# Autodesk Inventor assembly: Assembly_4_turnsignal_MIR
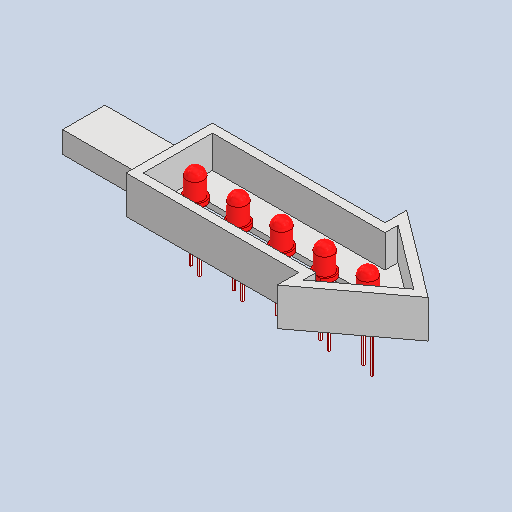
[picture p0: Inventor's stored thumbnail of the model, 512x512]
Saved by Autodesk Inventor 2023 (Build 270158000, 158)
## iProperties
Created: 2023-10-01
Part Number: Assembly_4_turnsignal_MIR
Document SubType Name: Assembly
Designer: zskus
Author: zskus
## Documents named in this file (3)
- C:\Users\zskus\Desktop\Folders\Personal Projects\Inventor\Project_1_Scooter\Assembly\Assembly_4_turnsignal_MIR.iam
- C:\Users\zskus\Desktop\Folders\Personal Projects\Inventor\Project_1_Scooter\Parts\Part_5_ledholder_MIR.ipt
- C:\Users\zskus\Desktop\Folders\Personal Projects\Inventor\Project_1_Scooter\Parts\red-led-5mm_MIR.ipt
## Components (6 placed, 2 different names)
1. Part_5_ledholder_MIR:1 — Mate:3, Mate:2, Mate:1
2. red-led-5mm_MIR:1 — Mate:3, Mate:2, Mate:1
3. red-led-5mm_MIR:2
4. red-led-5mm_MIR:3
5. red-led-5mm_MIR:4
6. red-led-5mm_MIR:5
## Component patterns: (5 elements, first: red-led-5mm_MIR:1)
## Relationships (3: Mate 3)
- Mate:3: Part_5_ledholder_MIR:1 ↔ red-led-5mm_MIR:1
- Mate:2: Part_5_ledholder_MIR:1 ↔ red-led-5mm_MIR:1
- Mate:1: Part_5_ledholder_MIR:1 ↔ red-led-5mm_MIR:1
